# Autodesk Inventor assembly: Yassembly
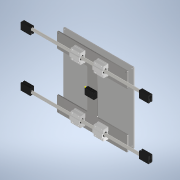
[picture p0: Inventor's stored thumbnail of the model, 180x180]
Saved by Autodesk Inventor 2020.2 (Build 242310000, 310)
## iProperties
Created: 2020-07-30
Part Number: Yassembly
Document SubType Name: Assembly
Designer: JK
Author: JK
## Documents named in this file (9)
- C:\Users\JK\Documents\Inventor\Anet Upgrade\Yassembly.iam
- C:\Users\JK\Documents\Inventor\Anet Upgrade\ycarriage.ipt
- C:\Users\JK\Documents\Inventor\Anet Upgrade\originalbed.ipt
- C:\Users\JK\Documents\Inventor\Anet Upgrade\LinearBearing8mm.iam
- C:\Users\JK\Documents\Inventor\Anet Upgrade\8x380axis.ipt
- C:\Users\JK\Documents\Inventor\Anet Upgrade\YsupportA.ipt
- C:\Users\JK\Documents\Inventor\Anet Upgrade\YsupportB.ipt
- C:\Users\JK\Documents\Inventor\Anet Upgrade\Y Belt Attachment A.ipt
- C:\Users\JK\Documents\Inventor\Anet Upgrade\Y Belt Attachment B.ipt
## Components (14 placed, 8 different names)
1. ycarriage:1 — Mate:1, Flush:1, Mate:9, Mate:10, Mate:11, Mate:12, Mate:14, Mate:15, Mate:16, Mate:25, Angle:1, Mate:26
2. originalbed:1 — Mate:1, Flush:1, Mate:9
3. LinearBearing8mm:1 [sub-assembly] — Flush:5, Flush:6, Flush:8, Mate:14, Mate:18
4. LinearBearing8mm:2 [sub-assembly] — Flush:5, Mate:16, Flush:9
5. LinearBearing8mm:3 [sub-assembly] — Flush:6, Flush:7, Mate:13, Mate:15, Flush:9
6. LinearBearing8mm:4 [sub-assembly] — Flush:7, Mate:10, Mate:11, Mate:12, Mate:13, Flush:8, Mate:17
7. Wał:1 — Mate:18, Flush:10, Mate:19, Mate:20, Mate:24
8. Wał:2 — Mate:17, Flush:10, Mate:21, Mate:22, Mate:23
9. YsupportA:1 — Mate:19, Mate:20, Flush:11, Flush:12, Flush:13
10. YsupportA:2 — Mate:21, Mate:22, Flush:11, Flush:14, Flush:15
11. YsupportB:1 — Mate:23, Flush:12, Flush:13
12. YsupportB:2 — Mate:24, Flush:14, Flush:15
13. Y Belt Attachment A:1 — Mate:25, Angle:1, Mate:26, Mate:27, Mate:28, Mate:29
14. Y Belt Attachment B:1 — Mate:27, Mate:28, Mate:29
## Relationships (35: Mate 22, Flush 12, Angle 1)
- Mate:1: ycarriage:1 ↔ originalbed:1
- Flush:1: ycarriage:1 ↔ originalbed:1
- Mate:9 (17 mm): ycarriage:1 ↔ originalbed:1
- Flush:5: LinearBearing8mm:1 ↔ LinearBearing8mm:2
- Flush:6: LinearBearing8mm:1 ↔ LinearBearing8mm:3
- Flush:7: LinearBearing8mm:3 ↔ LinearBearing8mm:4
- Mate:10: ycarriage:1 ↔ LinearBearing8mm:4
- Mate:11: ycarriage:1 ↔ LinearBearing8mm:4
- Mate:12: ycarriage:1 ↔ LinearBearing8mm:4
- Mate:13: LinearBearing8mm:3 ↔ LinearBearing8mm:4
- Flush:8: LinearBearing8mm:1 ↔ LinearBearing8mm:4
- Mate:14: ycarriage:1 ↔ LinearBearing8mm:1
- Mate:15: ycarriage:1 ↔ LinearBearing8mm:3
- Mate:16: ycarriage:1 ↔ LinearBearing8mm:2
- Flush:9: LinearBearing8mm:2 ↔ LinearBearing8mm:3
- Mate:17: LinearBearing8mm:4 ↔ Wał:2
- Mate:18: LinearBearing8mm:1 ↔ Wał:1
- Flush:10: Wał:1 ↔ Wał:2
- Mate:19: Wał:1 ↔ YsupportA:1
- Mate:20: Wał:1 ↔ YsupportA:1
- Mate:21: Wał:2 ↔ YsupportA:2
- Mate:22: Wał:2 ↔ YsupportA:2
- Flush:11: YsupportA:1 ↔ YsupportA:2
- Mate:23: Wał:2 ↔ YsupportB:1
- Flush:12: YsupportA:1 ↔ YsupportB:1
- Flush:13: YsupportA:1 ↔ YsupportB:1
- Mate:24: Wał:1 ↔ YsupportB:2
- Flush:14: YsupportA:2 ↔ YsupportB:2
- Flush:15: YsupportA:2 ↔ YsupportB:2
- Mate:25: ycarriage:1 ↔ Y Belt Attachment A:1
- Angle:1 (0 deg): ycarriage:1 ↔ Y Belt Attachment A:1
- Mate:26: ycarriage:1 ↔ Y Belt Attachment A:1
- Mate:27: Y Belt Attachment A:1 ↔ Y Belt Attachment B:1
- Mate:28: Y Belt Attachment A:1 ↔ Y Belt Attachment B:1
- Mate:29 (0.8 mm): Y Belt Attachment A:1 ↔ Y Belt Attachment B:1
